# Autodesk Inventor assembly: Control manifold
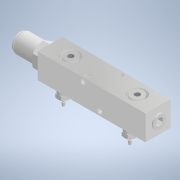
[picture p0: Inventor's stored thumbnail of the model, 180x180]
Saved by Autodesk Inventor 2021.2 (Build 252289000, 289)
## iProperties
Created: 2021-08-12
Part Number: Control manifold
Document SubType Name: Assembly
Designer: jl4459
Author: jl4459
## Documents named in this file (5)
- C:\Users\jl4459\Documents\Inventor\Training mini VR rig\Modules\Air puffs\Control manifold.iam
- C:\Users\jl4459\Documents\Inventor\Training mini VR rig\Modules\Air puffs\Parts\Manifold for gems solenoid valve vertical.ipt
- C:\Users\jl4459\Documents\Inventor\Training mini VR rig\Modules\Air puffs\Parts\1162T370_ZINC PLATED STEEL FITTINGS WITH SEALANT.ipt
- C:\Users\jl4459\Documents\Inventor\Training mini VR rig\Modules\Air puffs\Parts\2844K110_NICKEL-PLTD BRASS BARBED VACUUM TUBE FITTING.ipt
- C:\Users\jl4459\Documents\Inventor\Training mini VR rig\Modules\Air puffs\Parts\5779K115_PUSH-TO-CONNECT TUBE FITTING FOR AIR.ipt
## Components (5 placed, 4 different names)
1. Manifold for gems solenoid valve vertical:1 — Insert:1, Insert:2, Insert:3, Insert:4
2. 1162T370_ZINC PLATED STEEL FITTINGS WITH SEALANT:1 — Insert:1
3. 2844K110_NICKEL-PLTD BRASS BARBED VACUUM TUBE FITTING:1 — Insert:3
4. 2844K110_NICKEL-PLTD BRASS BARBED VACUUM TUBE FITTING:2 — Insert:2
5. 5779K115_PUSH-TO-CONNECT TUBE FITTING FOR AIR:1 — Insert:4
## Relationships (4: Insert 4)
- Insert:1 (-6.35 mm): Manifold for gems solenoid valve vertical:1 ↔ 1162T370_ZINC PLATED STEEL FITTINGS WITH SEALANT:1
- Insert:2: Manifold for gems solenoid valve vertical:1 ↔ 2844K110_NICKEL-PLTD BRASS BARBED VACUUM TUBE FITTING:2
- Insert:3: Manifold for gems solenoid valve vertical:1 ↔ 2844K110_NICKEL-PLTD BRASS BARBED VACUUM TUBE FITTING:1
- Insert:4 (-6.35 mm): Manifold for gems solenoid valve vertical:1 ↔ 5779K115_PUSH-TO-CONNECT TUBE FITTING FOR AIR:1
